# Autodesk Inventor assembly: GBX-900.1-grobox-casing
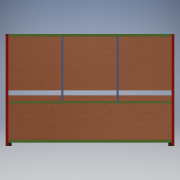
[picture p0: Inventor's stored thumbnail of the model, 180x180]
Saved by Autodesk Inventor 2019 (Build 230136000, 136)
## iProperties
Created: 2019-08-15
Part Number: GBX-900.1-grobox-casing
Document SubType Name: Assembly
Designer: Rene
Author: Rene
## Documents named in this file (9)
- C:\dev\c-scape\hardponics\dwg\grobox\GBX-900.1-grobox-casing.iam
- C:\dev\c-scape\hardponics\dwg\grobox\GBX_002.1-bottom-plate.ipt
- C:\dev\c-scape\hardponics\dwg\grobox\GBX_001.1-side-plate.ipt
- C:\dev\c-scape\hardponics\dwg\grobox\GBX_003.1-top-plate.ipt
- C:\dev\c-scape\hardponics\dwg\grobox\GBX_004.1-middle-plate.ipt
- C:\dev\c-scape\hardponics\dwg\grobox\GBX_005.1-fence-plate.ipt
- C:\dev\c-scape\hardponics\dwg\grobox\GBX_006.1-backplate_lo.ipt
- C:\dev\c-scape\hardponics\dwg\grobox\GBX_007.1-backplate_hi.ipt
- C:\dev\c-scape\hardponics\dwg\grobox\GBX_010.1-latje_15x15x300.ipt
## Components (11 placed, 8 different names)
1. GBX_002.1-bottom-plate:1 — Mate:1, Flush:1, Flush:2, Mate:2, Flush:3, Flush:4, Flush:17, Mate:20
2. GBX_001.1-side-plate:1 — Mate:1, Flush:1, Flush:2, Mate:3, Flush:6, Mate:9, Mate:23
3. GBX_001.1-side-plate:2 — Mate:2, Flush:3, Flush:4, Mate:4, Mate:7, Flush:13, Mate:14, Flush:14, Mate:19, Mate:24
4. GBX_003.1-top-plate:1 — Mate:3, Flush:6, Mate:5, Flush:13, Mate:17, Mate:21, Mate:22, Flush:18, Flush:19
5. GBX_004.1-middle-plate:1 — Mate:4, Mate:5, Mate:6, Mate:8, Mate:18, Flush:15, Flush:16
6. GBX_005.1-fence-plate:1 — Mate:8, Mate:9, Flush:16
7. GBX_005.1-fence-plate:2 — Mate:6, Mate:7, Flush:15
8. GBX_006.1-backplate_lo:1 — Mate:14, Mate:17, Flush:14, Mate:18
9. GBX_007.1-backplate_hi:1 — Flush:17, Mate:19, Mate:20
10. GBX_010.1-latje_15x15x300:1 — Mate:22, Mate:23, Flush:18
11. GBX_010.1-latje_15x15x300:2 — Mate:21, Mate:24, Flush:19
## Relationships (30: Mate 18, Flush 12)
- Mate:1: GBX_002.1-bottom-plate:1 ↔ GBX_001.1-side-plate:1
- Flush:1: GBX_002.1-bottom-plate:1 ↔ GBX_001.1-side-plate:1
- Flush:2: GBX_002.1-bottom-plate:1 ↔ GBX_001.1-side-plate:1
- Mate:2: GBX_002.1-bottom-plate:1 ↔ GBX_001.1-side-plate:2
- Flush:3: GBX_002.1-bottom-plate:1 ↔ GBX_001.1-side-plate:2
- Flush:4: GBX_002.1-bottom-plate:1 ↔ GBX_001.1-side-plate:2
- Mate:3: GBX_001.1-side-plate:1 ↔ GBX_003.1-top-plate:1
- Flush:6 (15 mm): GBX_001.1-side-plate:1 ↔ GBX_003.1-top-plate:1
- Mate:4: GBX_001.1-side-plate:2 ↔ GBX_004.1-middle-plate:1
- Mate:5 (156 mm): GBX_003.1-top-plate:1 ↔ GBX_004.1-middle-plate:1
- Mate:6: GBX_004.1-middle-plate:1 ↔ GBX_005.1-fence-plate:2
- Mate:7 (227.3333 mm): GBX_001.1-side-plate:2 ↔ GBX_005.1-fence-plate:2
- Mate:8: GBX_004.1-middle-plate:1 ↔ GBX_005.1-fence-plate:1
- Mate:9 (227.3333 mm): GBX_001.1-side-plate:1 ↔ GBX_005.1-fence-plate:1
- Flush:13: GBX_001.1-side-plate:2 ↔ GBX_003.1-top-plate:1
- Mate:14: GBX_001.1-side-plate:2 ↔ GBX_006.1-backplate_lo:1
- Mate:17: GBX_003.1-top-plate:1 ↔ GBX_006.1-backplate_lo:1
- Flush:14 (15 mm): GBX_001.1-side-plate:2 ↔ GBX_006.1-backplate_lo:1
- Mate:18: GBX_004.1-middle-plate:1 ↔ GBX_006.1-backplate_lo:1
- Flush:15: GBX_004.1-middle-plate:1 ↔ GBX_005.1-fence-plate:2
- Flush:16: GBX_004.1-middle-plate:1 ↔ GBX_005.1-fence-plate:1
- Flush:17 (15 mm): GBX_002.1-bottom-plate:1 ↔ GBX_007.1-backplate_hi:1
- Mate:19: GBX_001.1-side-plate:2 ↔ GBX_007.1-backplate_hi:1
- Mate:20: GBX_002.1-bottom-plate:1 ↔ GBX_007.1-backplate_hi:1
- Mate:21: GBX_003.1-top-plate:1 ↔ GBX_010.1-latje_15x15x300:2
- Mate:22: GBX_003.1-top-plate:1 ↔ GBX_010.1-latje_15x15x300:1
- Mate:23: GBX_001.1-side-plate:1 ↔ GBX_010.1-latje_15x15x300:1
- Mate:24: GBX_001.1-side-plate:2 ↔ GBX_010.1-latje_15x15x300:2
- Flush:18 (35 mm): GBX_003.1-top-plate:1 ↔ GBX_010.1-latje_15x15x300:1
- Flush:19 (35 mm): GBX_003.1-top-plate:1 ↔ GBX_010.1-latje_15x15x300:2
